# Autodesk Inventor assembly: outer
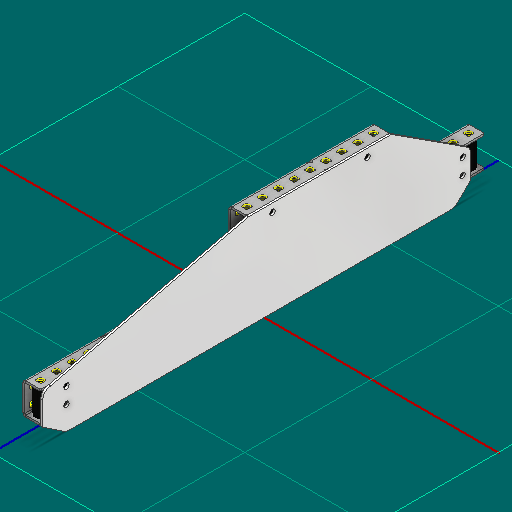
[picture p0: Inventor's stored thumbnail of the model, 512x512]
Saved by Autodesk Inventor 2025 (Build 290162000, 162)
## iProperties
Created: 2024-08-23
Part Number: outer
Document SubType Name: Assembly
Designer: averey
Author: averey
## Documents named in this file (8)
- C:\Users\avere\vex_robotics_high_stakes\hardware\cad\bots\CRAY-1\chassis\drivetrain\drivebay\outer.iam
- C:\Users\avere\vex_robotics_high_stakes\hardware\cad\VEX-CAD-Inventor\Structure\C Channel\Aluminum 1x2x1\Alu C 1x2x1x28.ipt
- C:\Users\avere\vex_robotics_high_stakes\hardware\cad\VEX-CAD-Inventor\Motion\Spacers\Spacer Nylon .375 OD\NSpacer .375 OD x .875.ipt
- C:\Users\avere\vex_robotics_high_stakes\hardware\cad\VEX-CAD-Inventor\Motion\Spacers\Spacer Nylon .375 OD.ipt
- C:\Users\avere\vex_robotics_high_stakes\hardware\cad\VEX-CAD-Inventor\Motion\Spacers\Spacer Nylon .500 OD\NSpacer White .500 OD x .500.ipt
- C:\Users\avere\vex_robotics_high_stakes\hardware\cad\VEX-CAD-Inventor\Motion\Spacers\Spacer Nylon .500 OD.ipt
- C:\Users\avere\vex_robotics_high_stakes\hardware\cad\VEX-CAD-Inventor\Structure\C Channel\Aluminum 1x2x1\Alu C 1x2x1x9.ipt
- C:\Users\avere\vex_robotics_high_stakes\hardware\cad\bots\CRAY-1\chassis\drivetrain\drivebay\custom_parts\skirt.ipt
## Components (7 placed, 5 different names)
1. NSpacer White .500 OD x .500:1 — Insert:3, Mate:3
2. NSpacer White .500 OD x .500:2 — Insert:4, Insert:5
3. Alu C 1x2x1x9:1 — Insert:5, Mate:3
4. skirt:1 — Insert:6, Mate:4
5. C-Channel — Flush:1, Mate:1, Mate:2, Insert:1, Insert:2, Insert:3, Insert:4, Insert:6, Mate:4
6. NSpacer .375 OD x .875:2 — Insert:2
7. NSpacer .375 OD x .875:1 — Insert:1
## Relationships (11: Insert 6, Mate 4, Flush 1)
- Flush:1 (-177.8 mm): C-Channel
- Mate:1: C-Channel
- Mate:2 (15.875 mm): C-Channel
- Insert:1: C-Channel ↔ NSpacer .375 OD x .875:1
- Insert:2: C-Channel ↔ NSpacer .375 OD x .875:2
- Insert:3: NSpacer White .500 OD x .500:1 ↔ C-Channel
- Insert:4: NSpacer White .500 OD x .500:2 ↔ C-Channel
- Insert:5: NSpacer White .500 OD x .500:2 ↔ Alu C 1x2x1x9:1
- Mate:3: NSpacer White .500 OD x .500:1 ↔ Alu C 1x2x1x9:1
- Insert:6 (12.7 mm): skirt:1 ↔ C-Channel
- Mate:4: skirt:1 ↔ C-Channel
